# Autodesk Inventor assembly: LowerBody
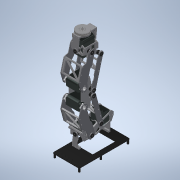
[picture p0: Inventor's stored thumbnail of the model, 180x180]
Saved by Autodesk Inventor 2020 (Build 240168000, 168)
## iProperties
Created: 2016-08-23
Part Number: LowerBody
Material: 一般
Document SubType Name: Assembly
Designer: hiro
Mass: 982.556 g
Surface Area: 2608.59 cm^2
Volume: 455.691 cm^3
Density: 2.15619 g/cm^3
Author: hiro
## Documents named in this file (12)
- C:\Users\naoki\Documents\Inventor\CitBrains\git_clone\OpenPlatform167\脚大改良後\OpenPlatform_ver3_0\LowerBody.iam
- C:\Users\naoki\Documents\Inventor\CitBrains\git_clone\OpenPlatform167\脚大改良後\OpenPlatform_ver3_0\下半身\足首\足首_1.iam
- C:\Users\naoki\Documents\Inventor\CitBrains\git_clone\OpenPlatform167\脚大改良後\OpenPlatform_ver3_0\下半身\足首\足首_独立ピッチ_1.iam
- C:\Users\naoki\Documents\Inventor\CitBrains\git_clone\OpenPlatform167\脚大改良後\OpenPlatform_ver3_0\下半身\リンク\LowerFrontLink.iam
- C:\Users\naoki\Documents\Inventor\CitBrains\git_clone\OpenPlatform167\脚大改良後\OpenPlatform_ver3_0\下半身\付け根ロール\付け根ロール_1.iam
- C:\Users\naoki\Documents\Inventor\CitBrains\git_clone\OpenPlatform167\脚大改良後\OpenPlatform_ver3_0\下半身\リンク\LowerBackLink.iam
- C:\Users\naoki\Documents\Inventor\CitBrains\git_clone\OpenPlatform167\脚大改良後\OpenPlatform_ver3_0\下半身\長穴減速\長穴減速_ホーン.iam
- C:\Users\naoki\Documents\Inventor\CitBrains\git_clone\OpenPlatform167\脚大改良後\OpenPlatform_ver3_0\下半身\膝\膝_1.iam
- C:\Users\naoki\Documents\Inventor\CitBrains\git_clone\OpenPlatform167\脚大改良後\OpenPlatform_ver3_0\下半身\付け根\付け根_1.iam
- C:\Users\naoki\Documents\Inventor\CitBrains\git_clone\OpenPlatform167\脚大改良後\OpenPlatform_ver3_0\下半身\リンク\UpperBackLink.iam
- C:\Users\naoki\Documents\Inventor\CitBrains\git_clone\OpenPlatform167\脚大改良後\OpenPlatform_ver3_0\下半身\リンク\UpperFrontLink.iam
- C:\Users\naoki\Documents\Inventor\CitBrains\git_clone\OpenPlatform167\脚大改良後\OpenPlatform_ver3_0\下半身\足裏\foot.iam
## Components (12 placed, 11 different names)
1. 付け根ロール_1:1 [sub-assembly] — 角度:4, 角度:8, 角度:12, フラッシュ:4, 挿入:146, 挿入:147
2. 長穴減速_ホーン:1 [sub-assembly] — 挿入:145, 挿入:146
3. 付け根_1:1 [sub-assembly] — 角度:4, メイト:1, メイト:2, 挿入:142, 挿入:144, 挿入:145, 挿入:147
4. UpperFrontLink:1 [sub-assembly] — 角度:12, 挿入:139, 挿入:144
5. UpperBackLink:1 [sub-assembly] — 挿入:141, 挿入:142
6. 膝_1:1 [sub-assembly] — 挿入:129, 挿入:139, 挿入:141, 挿入:143
7. LowerFrontLink:2 [sub-assembly] — 角度:11, 挿入:129, 挿入:148
8. LowerBackLink:1 [sub-assembly] — 挿入:143, 挿入:149, 挿入:151
9. 足首_1:1 [sub-assembly] — 挿入:117, 挿入:124, 挿入:150
10. Foot:1 [sub-assembly] — 角度:8, 挿入:117, 角度:11
11. 足首_独立ピッチ_1:1 [sub-assembly] — 挿入:124, 挿入:148, 挿入:149
12. 足首_独立ピッチ_1:2 [sub-assembly] — 挿入:150, 挿入:151
## Relationships (22: Insert 15, Angle 4, Mate 2, Flush 1)
- 角度:4 [Angle] (0 deg): 付け根ロール_1:1 ↔ 付け根_1:1
- 角度:8 [Angle] (0 deg): 付け根ロール_1:1 ↔ Foot:1
- 挿入:117 [Insert]: 足首_1:1 ↔ Foot:1
- 角度:11 [Angle] (15 deg): LowerFrontLink:2 ↔ Foot:1
- 角度:12 [Angle] (15 deg): 付け根ロール_1:1 ↔ UpperFrontLink:1
- 挿入:124 [Insert]: 足首_1:1 ↔ 足首_独立ピッチ_1:1
- 挿入:129 [Insert]: 膝_1:1 ↔ LowerFrontLink:2
- メイト:1 [Mate] (-16.5 mm): 付け根_1:1
- メイト:2 [Mate] (-27 mm): 付け根_1:1
- フラッシュ:4 [Flush]: 付け根ロール_1:1
- 挿入:139 [Insert]: UpperFrontLink:1 ↔ 膝_1:1
- 挿入:141 [Insert]: UpperBackLink:1 ↔ 膝_1:1
- 挿入:142 [Insert]: 付け根_1:1 ↔ UpperBackLink:1
- 挿入:143 [Insert]: 膝_1:1 ↔ LowerBackLink:1
- 挿入:144 [Insert]: 付け根_1:1 ↔ UpperFrontLink:1
- 挿入:145 [Insert]: 長穴減速_ホーン:1 ↔ 付け根_1:1
- 挿入:146 [Insert]: 付け根ロール_1:1 ↔ 長穴減速_ホーン:1
- 挿入:147 [Insert]: 付け根ロール_1:1 ↔ 付け根_1:1
- 挿入:148 [Insert]: LowerFrontLink:2 ↔ 足首_独立ピッチ_1:1
- 挿入:149 [Insert]: LowerBackLink:1 ↔ 足首_独立ピッチ_1:1
- 挿入:150 [Insert]: 足首_1:1 ↔ 足首_独立ピッチ_1:2
- 挿入:151 [Insert]: LowerBackLink:1 ↔ 足首_独立ピッチ_1:2
